# Autodesk Inventor assembly: projeto de escada de aço padrão
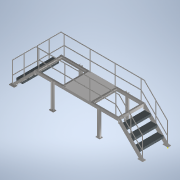
[picture p0: Inventor's stored thumbnail of the model, 180x180]
Saved by Autodesk Inventor 2022 (Build 260153000, 153)
## iProperties
Created: 2021-11-17
Part Number: projeto de escada de aço padrão
Document SubType Name: Assembly
Designer: FlavianyVieiraMagesc
Author: FlavianyVieiraMagesc
## Documents named in this file (6)
- D:\Area de Trabalho\PROJETOS\arquivos inventor\mini grua\plataforma\projeto de escada de aço padrão.iam
- D:\Area de Trabalho\PROJETOS\arquivos inventor\mini grua\plataforma\Frame Wire.ipt
- D:\Area de Trabalho\PROJETOS\arquivos inventor\mini grua\plataforma\projeto de escada de aço padrão\Frame\Quadro estrutural.iam
- D:\Area de Trabalho\PROJETOS\arquivos inventor\mini grua\plataforma\Step.ipt
- D:\Area de Trabalho\PROJETOS\arquivos inventor\mini grua\plataforma\Step_MIR.ipt
- D:\Area de Trabalho\PROJETOS\arquivos inventor\mini grua\plataforma\Plate.ipt
## Components (9 placed, 5 different names)
1. Frame Wire:1 — Alinhado:1
2. Quadro estrutural:1 [sub-assembly] — Alinhado:2, Alinhado:3, Alinhado:4, Alinhado:5, Alinhado:6
3. Step_MIR:1
4. Step_MIR:2
5. Step_MIR:3
6. Plate:1 — Alinhado:5, Alinhado:6
7. Step:1 — Alinhado:2, Alinhado:3, Alinhado:4
8. Step:2
9. Step:3
## Component patterns: (3 elements, first: Step:1)
## Relationships (6: Flush 6)
- Alinhado:1 [Flush]: Frame Wire:1
- Alinhado:2 [Flush]: Quadro estrutural:1 ↔ Step:1
- Alinhado:3 [Flush]: Quadro estrutural:1 ↔ Step:1
- Alinhado:4 [Flush]: Quadro estrutural:1 ↔ Step:1
- Alinhado:5 [Flush]: Quadro estrutural:1 ↔ Plate:1
- Alinhado:6 [Flush]: Quadro estrutural:1 ↔ Plate:1
